# Autodesk Inventor assembly: pist
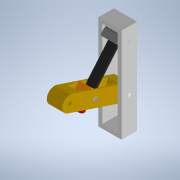
[picture p0: Inventor's stored thumbnail of the model, 180x180]
Saved by Autodesk Inventor 2022 (Build 260153000, 153)
## iProperties
Created: 2022-11-09
Part Number: pist
Document SubType Name: Assembly
Designer: matys
Author: matys
## Documents named in this file (9)
- C:\Users\matys\Desktop\Práce4tak\Inventor\mechanismus odpruzeni\pist.iam
- C:\Users\matys\Desktop\Práce4tak\Inventor\mechanismus odpruzeni\pist-zatka.ipt
- C:\Users\matys\Desktop\Práce4tak\Inventor\mechanismus odpruzeni\pist.ipt
- C:\Users\matys\Desktop\Práce4tak\Inventor\mechanismus odpruzeni\top.ipt
- C:\Users\matys\Desktop\Práce4tak\Inventor\mechanismus odpruzeni\mid.ipt
- C:\Users\matys\Desktop\Práce4tak\Inventor\novy tank\tycinka.ipt
- C:\Users\matys\Desktop\Práce4tak\Inventor\mechanismus odpruzeni\pist-dolni.ipt
- C:\Users\matys\Desktop\Práce4tak\Inventor\novy tank\tycinka_12mm.ipt
- C:\Users\matys\Desktop\Práce4tak\Inventor\novy tank\spring.ipt
## Components (9 placed, 8 different names)
1. pist-zatka:1 — Mate:7, Mate:8, Mate:12
2. pist:1 — Mate:7, Mate:8, Mate:9, Mate:10, Mate:11, Mate:16, Mate:17
3. top:1 — Mate:1, Mate:2, Mate:3, Mate:4, Mate:6, Mate:10
4. mid:1 — Mate:5, Mate:6, Mate:14, Mate:15
5. tycinka:2 — Mate:3, Mate:4, Mate:5
6. tycinka:3 — Mate:1, Mate:2, Mate:9
7. pist-dolni:1 — Mate:11, Mate:12, Mate:13
8. tycinka_12mm:1 — Mate:13, Mate:14, Mate:15
9. spring:1 — Mate:16, Mate:17
## Relationships (17: Mate 17)
- Mate:1: top:1 ↔ tycinka:3
- Mate:2: top:1 ↔ tycinka:3
- Mate:3: top:1 ↔ tycinka:2
- Mate:4: top:1 ↔ tycinka:2
- Mate:5: mid:1 ↔ tycinka:2
- Mate:6: top:1 ↔ mid:1
- Mate:7: pist-zatka:1 ↔ pist:1
- Mate:8: pist-zatka:1 ↔ pist:1
- Mate:9: pist:1 ↔ tycinka:3
- Mate:10: pist:1 ↔ top:1
- Mate:11: pist:1 ↔ pist-dolni:1
- Mate:12: pist-zatka:1 ↔ pist-dolni:1
- Mate:13: pist-dolni:1 ↔ tycinka_12mm:1
- Mate:14: mid:1 ↔ tycinka_12mm:1
- Mate:15: mid:1 ↔ tycinka_12mm:1
- Mate:16: pist:1 ↔ spring:1
- Mate:17: pist:1 ↔ spring:1
